# Autodesk Inventor assembly: ASY ANP 1426 FDS way 6
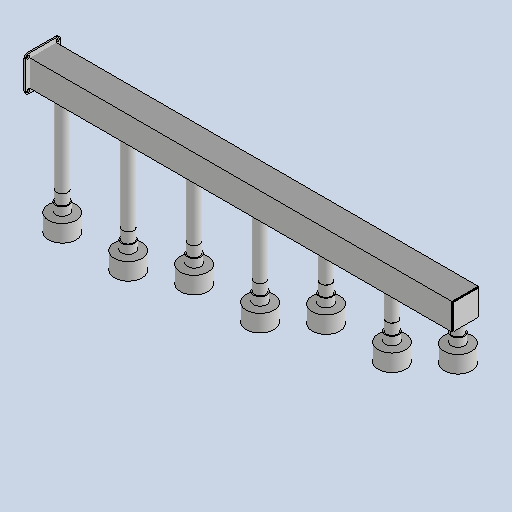
[picture p0: Inventor's stored thumbnail of the model, 512x512]
Saved by Autodesk Inventor 2025 (Build 290162010, 162A)
## iProperties
Created: 2025-07-02
Part Number: ASY ANP 1426 FDS way 6
Document SubType Name: Assembly
Designer: admin
Author: user
## Documents named in this file (9)
- C:\Users\admin\Yandex.Disk\home pc\Inventor\ANP--Antipayuta\FDS 1400\ASY ANP 1426 FDS way 6.iam
- C:\Users\admin\Yandex.Disk\home pc\Inventor\ANP--Antipayuta\FDS 1400\ANP 1436 FDS WAY tube6.ipt
- C:\Users\admin\Yandex.Disk\home pc\Inventor\ANP--Antipayuta\FDS 1400\ANP 1425 FDS Way FLANGE.ipt
- C:\Users\admin\Yandex.Disk\home pc\Inventor\ANP--Antipayuta\FDS 1400\ANP 1426 FDS way cup.ipt
- C:\Users\admin\Yandex.Disk\home pc\Inventor\ANP--Antipayuta\FDS 1400\ANP dummy filter element.ipt
- C:\Users\admin\Yandex.Disk\home pc\Inventor\ANP--Antipayuta\FDS 1400\ANP dummy pipe nippel.ipt
- C:\Users\admin\Yandex.Disk\home pc\Inventor\ANP--Antipayuta\FDS 1400\ANP 1448 FDS thread  tube8.ipt
- C:\Users\admin\Yandex.Disk\home pc\Inventor\ANP--Antipayuta\FDS 1400\ANP 1449 FDS thread  tube9.ipt
- C:\Users\admin\Yandex.Disk\home pc\Inventor\ANP--Antipayuta\FDS 1400\ANP 1451 FDS thread  tube10.ipt
## Components (23 placed, 8 different names)
1. ANP 1436 FDS WAY tube6.ipt:1 — Rigid:34, Rigid:35, Rigid:36, Rigid:53, Rigid:54, Rigid:55, Rigid:26, Rigid:27, Rigid:28
2. ANP 1425 FDS Way FLANGE.ipt:1 — Rigid:34
3. ANP 1426 FDS way cup.ipt:1 — Rigid:35
4. ANP dummy filter element.ipt:1 — Rigid:1
5. ANP dummy pipe nippel.ipt:1 — Rigid:1, Rigid:44
6. ANP dummy filter element.ipt:2 — Rigid:6
7. ANP dummy pipe nippel.ipt:2 — Rigid:6, Rigid:46
8. ANP dummy filter element.ipt:3 — Rigid:14
9. ANP dummy pipe nippel.ipt:3 — Rigid:14, Rigid:45
10. ANP dummy filter element.ipt:4 — Rigid:33
11. ANP dummy pipe nippel.ipt:4 — Rigid:36, Rigid:33
12. ANP 1448 FDS thread  tube8.ipt:1 — Rigid:53, Rigid:46
13. ANP 1449 FDS thread  tube9.ipt:1 — Rigid:54, Rigid:45
14. ANP 1451 FDS thread  tube10.ipt:1 — Rigid:55, Rigid:44
15. ANP dummy filter element.ipt:5
16. ANP dummy pipe nippel.ipt:5
17. ANP dummy filter element.ipt:6
18. ANP dummy pipe nippel.ipt:6
19. ANP 1448 FDS thread  tube8.ipt:2 — Rigid:28
20. ANP 1449 FDS thread  tube9.ipt:2 — Rigid:27
21. ANP dummy filter element.ipt:7
22. ANP dummy pipe nippel.ipt:7
23. ANP 1451 FDS thread  tube10.ipt:2 — Rigid:26
## Relationships (22: WeldJoint 22)
- Rigid:34 [WeldJoint] (2 mm): ANP 1436 FDS WAY tube6.ipt:1 ↔ ANP 1425 FDS Way FLANGE.ipt:1
- Rigid:35 [WeldJoint]: ANP 1436 FDS WAY tube6.ipt:1 ↔ ANP 1426 FDS way cup.ipt:1
- Rigid:1 [WeldJoint]: ANP dummy filter element.ipt:1 ↔ ANP dummy pipe nippel.ipt:1
- Rigid:6 [WeldJoint]: ANP dummy filter element.ipt:2 ↔ ANP dummy pipe nippel.ipt:2
- Rigid:14 [WeldJoint]: ANP dummy filter element.ipt:3 ↔ ANP dummy pipe nippel.ipt:3
- Rigid:36 [WeldJoint]: ANP 1436 FDS WAY tube6.ipt:1 ↔ ANP dummy pipe nippel.ipt:4
- Rigid:33 [WeldJoint]: ANP dummy filter element.ipt:4 ↔ ANP dummy pipe nippel.ipt:4
- Rigid:53 [WeldJoint]: ANP 1436 FDS WAY tube6.ipt:1 ↔ ANP 1448 FDS thread  tube8.ipt:1
- Rigid:46 [WeldJoint]: ANP dummy pipe nippel.ipt:2 ↔ ANP 1448 FDS thread  tube8.ipt:1
- Rigid:54 [WeldJoint]: ANP 1436 FDS WAY tube6.ipt:1 ↔ ANP 1449 FDS thread  tube9.ipt:1
- Rigid:45 [WeldJoint]: ANP dummy pipe nippel.ipt:3 ↔ ANP 1449 FDS thread  tube9.ipt:1
- Rigid:55 [WeldJoint]: ANP 1436 FDS WAY tube6.ipt:1 ↔ ANP 1451 FDS thread  tube10.ipt:1
- Rigid:44 [WeldJoint]: ANP dummy pipe nippel.ipt:1 ↔ ANP 1451 FDS thread  tube10.ipt:1
- [WeldJoint]: ANP dummy filter element.ipt:5 ↔ ANP dummy pipe nippel.ipt:5
- [WeldJoint]: ANP dummy filter element.ipt:6 ↔ ANP dummy pipe nippel.ipt:6
- [WeldJoint]: ANP dummy pipe nippel.ipt:5 ↔ ANP 1448 FDS thread  tube8.ipt:2
- [WeldJoint]: ANP dummy pipe nippel.ipt:6 ↔ ANP 1449 FDS thread  tube9.ipt:2
- [WeldJoint]: ANP dummy filter element.ipt:7 ↔ ANP dummy pipe nippel.ipt:7
- [WeldJoint]: ANP dummy pipe nippel.ipt:7 ↔ ANP 1451 FDS thread  tube10.ipt:2
- Rigid:26 [WeldJoint]: ANP 1436 FDS WAY tube6.ipt:1 ↔ ANP 1451 FDS thread  tube10.ipt:2
- Rigid:27 [WeldJoint]: ANP 1436 FDS WAY tube6.ipt:1 ↔ ANP 1449 FDS thread  tube9.ipt:2
- Rigid:28 [WeldJoint]: ANP 1436 FDS WAY tube6.ipt:1 ↔ ANP 1448 FDS thread  tube8.ipt:2
## Named parameters: d25_d14 = 0 mm, d26_d16 = 0 mm, d27_d3 = 0 mm, d28_d5 = 0 mm, d29_d18 = 0 mm, d30_d2 = 0 mm
